# Autodesk Inventor assembly: holder_with_battery
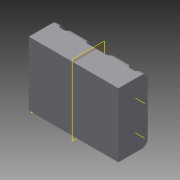
[picture p0: Inventor's stored thumbnail of the model, 180x180]
Saved by Autodesk Inventor 2014 (Build 180170000, 170)
## iProperties
Created: 2013-06-25
Part Number: holder_with_battery
Document SubType Name: Assembly
Designer: Felix
Author: Felix
## Documents named in this file (3)
- C:\Users\Felix\Desktop\Robot\battery_holder\holder_with_batteries.iam
- C:\Users\Felix\Desktop\Robot\battery_holder\battery_18500.ipt
- C:\Users\Felix\Desktop\Robot\battery_holder\holder.ipt
## Components (3 placed, 3 different names)
1. battery_18500:1 — Passend:1
2. holder:1 — Passend:1, Passend:2
3. accu_18500:2 — Passend:2
## Relationships (2: Mate 2)
- Passend:1 [Mate]: battery_18500:1 ↔ holder:1
- Passend:2 [Mate]: holder:1 ↔ accu_18500:2
